# Autodesk Inventor assembly: Orbbec Astra
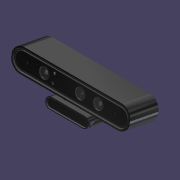
[picture p0: Inventor's stored thumbnail of the model, 180x180]
Saved by Autodesk Inventor 2017 SP1 (Build 210196100, 196)
## iProperties
Created: 2018-05-26
Part Number: Orbbec Astra
Document SubType Name: Assembly
Designer: Zach
Author: Zach
## iProperties of the stored document Mount_Part2.ipt
Created: 2017-11-22
Part Number: Mount_Part2
Material: Generic
Document SubType Name: Modeling
Designer: Zach
Density: 1 g/cm^3
Appearance: Default
Sending System: SolidWorks 2016
Last Author: tgv
Last Saved: 2017-12-01
Author: Zach
## iProperties of the stored document MainBody.ipt
Created: 2017-11-22
Part Number: MainBody
Material: Generic
Document SubType Name: Modeling
Designer: Zach
Density: 1 g/cm^3
Appearance: Default
Sending System: SolidWorks 2016
Last Author: tgv
Last Saved: 2017-12-01
Author: Zach
## iProperties of the stored document Main_Body.iam
Created: 2017-11-22
Part Number: Main_Body
Document SubType Name: Assembly
Designer: Zach
Sending System: SolidWorks 2016
Last Author: tgv
Last Saved: 2017-12-01
Author: Zach
## iProperties of the stored document Mount_Part1.ipt
Created: 2017-11-22
Part Number: Mount_Part1
Material: Generic
Document SubType Name: Modeling
Designer: Zach
Density: 1 g/cm^3
Appearance: Default
Sending System: SolidWorks 2016
Last Author: tgv
Last Saved: 2017-12-01
Author: Zach
## iProperties of the stored document SGlass1.ipt
Created: 2017-11-22
Part Number: SGlass1
Material: Generic
Document SubType Name: Modeling
Designer: Zach
Density: 1 g/cm^3
Appearance: Default
Sending System: SolidWorks 2016
Last Author: tgv
Last Saved: 2017-12-01
Author: Zach
## iProperties of the stored document Glass1.ipt
Created: 2017-11-22
Part Number: Glass1
Material: Generic
Document SubType Name: Modeling
Designer: Zach
Density: 1 g/cm^3
Appearance: Default
Sending System: SolidWorks 2016
Last Author: tgv
Last Saved: 2017-12-01
Author: Zach
## Documents named in this file (13)
- C:\Users\Zach\Documents\GitHub\tr1\lib\Orbbec Astra\Orbbec Astra.iam
- **C:\Users\Zach\Documents\GitHub\tr1\lib\Orbbec Astra\Orbbec Astra.iam*LocalDocs*xS2adnwq0Mimluu0wH01zfqzqZh*Mount_Part1.ipt
- **C:\Users\Zach\Documents\GitHub\tr1\lib\Orbbec Astra\Orbbec Astra.iam*LocalDocs*xElyp5v5b0wsdeooyQ03kmh42Dg*Mount_Part2.ipt
- **C:\Users\Zach\Documents\GitHub\tr1\lib\Orbbec Astra\Orbbec Astra.iam*LocalDocs*xSap12iecH52xuzcaCjiv0nkwYb*Main_Body.iam
- **C:\Users\Zach\Documents\GitHub\tr1\lib\Orbbec Astra\Orbbec Astra.iam*LocalDocs*x24qyujvrRg3culgwCmfwhqjo0h*MainBody.ipt
- **C:\Users\Zach\Documents\GitHub\tr1\lib\Orbbec Astra\Orbbec Astra.iam*LocalDocs*xXwyszjqlOlyxuxwx5daioaa5Tb*Glass1.ipt
- **C:\Users\Zach\Documents\GitHub\tr1\lib\Orbbec Astra\Orbbec Astra.iam*LocalDocs*xWl1hlrv5Aurkeo05WdijbyjfPg*SGlass1.ipt
- C:\Users\Zach\Documents\GitHub\tr1\lib\Orbbec Astra\Astra\Mount_Part1.sldprt
- C:\Users\Zach\Documents\GitHub\tr1\lib\Orbbec Astra\Astra\Mount_Part2.sldprt
- C:\Users\Zach\Documents\GitHub\tr1\lib\Orbbec Astra\Astra\Glass1.sldprt
- C:\Users\Zach\Documents\GitHub\tr1\lib\Orbbec Astra\Astra\MainBody.sldprt
- C:\Users\Zach\Documents\GitHub\tr1\lib\Orbbec Astra\Astra\Main_Body.sldasm
- C:\Users\Zach\Documents\GitHub\tr1\lib\Orbbec Astra\Astra\SGlass1.sldprt
## Components (3 placed, 3 different names)
1. Mount_Part1:1 — Mate:1, Mate:2, Mate:3, Mate:4, Angle:1, Angle:2
2. Mount_Part2:1 — Mate:2, Mate:4, Angle:2
3. Main_Body:1 [sub-assembly] — Mate:1, Mate:3, Angle:1
## Relationships (6: Mate 4, Angle 2)
- Mate:1: Mount_Part1:1 ↔ Main_Body:1
- Mate:2: Mount_Part1:1 ↔ Mount_Part2:1
- Mate:3 (0.1 mm): Mount_Part1:1 ↔ Main_Body:1
- Mate:4 (1 mm): Mount_Part1:1 ↔ Mount_Part2:1
- Angle:1 (0 deg): Mount_Part1:1 ↔ Main_Body:1
- Angle:2 (180 deg): Mount_Part1:1 ↔ Mount_Part2:1
